# Autodesk Inventor assembly: battery holder 3 x AAA
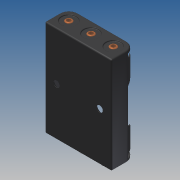
[picture p0: Inventor's stored thumbnail of the model, 180x180]
Saved by Autodesk Inventor 2012 SP1 (Build 160190100, 190)
## iProperties
Created: 2012-12-05
Part Number: battery holder 3 x AAA
Document SubType Name: Assembly
Designer: Komp
Author: Komp
## Documents named in this file (5)
- K:\tomek\backup 25.06\studia\CAD\battery holder 3 x AAA.iam
- K:\tomek\backup 25.06\studia\CAD\3x AAA battery holder.ipt
- K:\tomek\backup 25.06\studia\CAD\wstawka.ipt
- K:\tomek\backup 25.06\studia\CAD\sprężyna.ipt
- K:\tomek\backup 25.06\studia\CAD\wtyczka.ipt
## Components (12 placed, 4 different names)
1. 3x AAA battery holder:1 — Wstaw:1, Wstaw:2, Równoległy:2, Wstaw:3, Wstaw:4, Wstaw:5, Wstaw:6, Równoległy:5, Równoległy:7, Wstaw:7, Wstaw:8
2. wstawka:1 — Wstaw:2
3. wstawka:2 — Wstaw:1, Równoległy:1, Zestawiający:1
4. sprężyna:1 — Równoległy:1, Zestawiający:1, Równoległy:2
5. wstawka:3 — Wstaw:3, Równoległy:3, Równoległy:4
6. wstawka:4 — Wstaw:6
7. wstawka:5 — Wstaw:5, Równoległy:6, Zestawiający:2
8. wstawka:6 — Wstaw:4
9. sprężyna:2 — Równoległy:3, Równoległy:4, Równoległy:5
10. sprężyna:3 — Równoległy:6, Zestawiający:2, Równoległy:7
11. wtyczka:1 — Wstaw:7
12. wtyczka:2 — Wstaw:8
## Relationships (17: Insert 8, Flush 7, Mate 2)
- Wstaw:1 [Insert] (-0.2 mm): 3x AAA battery holder:1 ↔ wstawka:2
- Wstaw:2 [Insert] (-0.2 mm): 3x AAA battery holder:1 ↔ wstawka:1
- Równoległy:1 [Flush]: wstawka:2 ↔ sprężyna:1
- Zestawiający:1 [Mate]: wstawka:2 ↔ sprężyna:1
- Równoległy:2 [Flush]: 3x AAA battery holder:1 ↔ sprężyna:1
- Wstaw:3 [Insert] (-0.2 mm): 3x AAA battery holder:1 ↔ wstawka:3
- Wstaw:4 [Insert] (-0.2 mm): 3x AAA battery holder:1 ↔ wstawka:6
- Wstaw:5 [Insert] (-0.2 mm): 3x AAA battery holder:1 ↔ wstawka:5
- Wstaw:6 [Insert] (-0.2 mm): 3x AAA battery holder:1 ↔ wstawka:4
- Równoległy:3 [Flush]: wstawka:3 ↔ sprężyna:2
- Równoległy:4 [Flush]: wstawka:3 ↔ sprężyna:2
- Równoległy:5 [Flush]: 3x AAA battery holder:1 ↔ sprężyna:2
- Równoległy:6 [Flush]: wstawka:5 ↔ sprężyna:3
- Zestawiający:2 [Mate]: wstawka:5 ↔ sprężyna:3
- Równoległy:7 [Flush]: 3x AAA battery holder:1 ↔ sprężyna:3
- Wstaw:7 [Insert]: 3x AAA battery holder:1 ↔ wtyczka:1
- Wstaw:8 [Insert]: 3x AAA battery holder:1 ↔ wtyczka:2
